# Autodesk Inventor assembly: Assembly 1
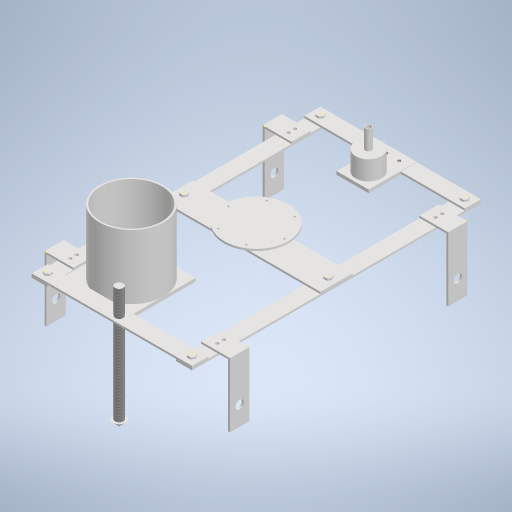
[picture p0: Inventor's stored thumbnail of the model, 512x512]
Saved by Autodesk Inventor 2024 (Build 280153000, 153)
## iProperties
Created: 2024-02-06
Part Number: Assembly 1
Document SubType Name: Assembly
Designer: Ramji Yadav
Author: Ramji Yadav
## Documents named in this file (8)
- D:\B.Tech\2nd Year\4rth Sem\Academics\TA 212\Project Parts\Assembly 1.iam
- D:\B.Tech\2nd Year\4rth Sem\Academics\TA 212\Project Parts\Base Platform.ipt
- D:\B.Tech\2nd Year\4rth Sem\Academics\TA 212\Project Parts\Screw.ipt
- D:\B.Tech\2nd Year\4rth Sem\Academics\TA 212\Project Parts\Angle.ipt
- D:\B.Tech\2nd Year\4rth Sem\Academics\TA 212\Project Parts\Digging Tool.ipt
- D:\B.Tech\2nd Year\4rth Sem\Academics\TA 212\Project Parts\Center Lower Disk.ipt
- D:\B.Tech\2nd Year\4rth Sem\Academics\TA 212\Project Parts\Reservoir.ipt
- D:\B.Tech\2nd Year\4rth Sem\Academics\TA 212\Project Parts\Pump.ipt
## Components (15 placed, 7 different names)
1. Base Platform:1 — Mate:1, Mate:2, Mate:3, Mate:4, Mate:5, Mate:6, Mate:7, Mate:8, Mate:9, Mate:10, Mate:11, Mate:12, Mate:13, Mate:14, Mate:15, Mate:16, Mate:17, Mate:18, Mate:19, Mate:20, Mate:21, Mate:22, Mate:23, Mate:24, Mate:25, Mate:26, Mate:27, Mate:28, Mate:29, Mate:30, Mate:31, Mate:32, Mate:33
2. Screw:1 — Mate:1, Mate:2, Mate:3
3. Screw:2 — Mate:4, Mate:7
4. Screw:3 — Mate:5, Mate:6
5. Screw:4 — Mate:8, Mate:9
6. Screw:5 — Mate:10
7. Screw:6 — Mate:11, Mate:12
8. Angle:1 — Mate:13, Mate:14, Mate:15
9. Angle:2 — Mate:16, Mate:17, Mate:18, Mate:19
10. Angle:3 — Mate:20, Mate:21, Mate:22, Mate:23
11. Angle:4 — Mate:24, Mate:25, Mate:26, Mate:27
12. Digging Tool:1 — Mate:28
13. Center Lower Disk:1 — Mate:29
14. Reservoir:1 — Mate:30, Mate:31
15. Pump:1 — Mate:32, Mate:33
## Relationships (33: Mate 33)
- Mate:1 (50 mm): Base Platform:1 ↔ Screw:1
- Mate:2: Base Platform:1 ↔ Screw:1
- Mate:3: Base Platform:1 ↔ Screw:1
- Mate:4: Base Platform:1 ↔ Screw:2
- Mate:5: Base Platform:1 ↔ Screw:3
- Mate:6: Base Platform:1 ↔ Screw:3
- Mate:7: Base Platform:1 ↔ Screw:2
- Mate:8: Base Platform:1 ↔ Screw:4
- Mate:9: Base Platform:1 ↔ Screw:4
- Mate:10: Base Platform:1 ↔ Screw:5
- Mate:11: Base Platform:1 ↔ Screw:6
- Mate:12: Base Platform:1 ↔ Screw:6
- Mate:13: Base Platform:1 ↔ Angle:1
- Mate:14: Base Platform:1 ↔ Angle:1
- Mate:15: Base Platform:1 ↔ Angle:1
- Mate:16: Base Platform:1 ↔ Angle:2
- Mate:17: Base Platform:1 ↔ Angle:2
- Mate:18: Base Platform:1 ↔ Angle:2
- Mate:19: Base Platform:1 ↔ Angle:2
- Mate:20: Base Platform:1 ↔ Angle:3
- Mate:21: Base Platform:1 ↔ Angle:3
- Mate:22: Base Platform:1 ↔ Angle:3
- Mate:23: Base Platform:1 ↔ Angle:3
- Mate:24: Base Platform:1 ↔ Angle:4
- Mate:25: Base Platform:1 ↔ Angle:4
- Mate:26: Base Platform:1 ↔ Angle:4
- Mate:27: Base Platform:1 ↔ Angle:4
- Mate:28: Base Platform:1 ↔ Digging Tool:1
- Mate:29: Base Platform:1 ↔ Center Lower Disk:1
- Mate:30: Base Platform:1 ↔ Reservoir:1
- Mate:31: Base Platform:1 ↔ Reservoir:1
- Mate:32: Base Platform:1 ↔ Pump:1
- Mate:33: Base Platform:1 ↔ Pump:1
